# Autodesk Inventor assembly: test_rig_asmbly
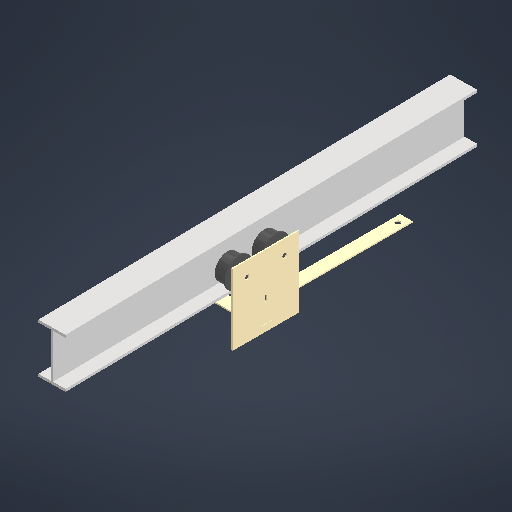
[picture p0: Inventor's stored thumbnail of the model, 512x512]
Saved by Autodesk Inventor 2027.1 (Build 311270010, 270A)
## iProperties
Created: 2026-09-04
Part Number: test_rig_asmbly
Document SubType Name: Assembly
Designer: ajrcr
Author: ajrcr
## Documents named in this file (6)
- C:\Users\ajrcr\OneDrive\Documents\Y3_s2\MCTR327\Git_Repo\Design-2026\3D parts\test_rig_asmbly.iam
- C:\Users\ajrcr\OneDrive\Documents\Y3_s2\MCTR327\Git_Repo\Design-2026\3D parts\Rail_beam.ipt
- C:\Users\ajrcr\OneDrive\Documents\Y3_s2\MCTR327\Git_Repo\Design-2026\3D parts\test_wheel_v1.ipt
- C:\Users\ajrcr\OneDrive\Documents\Y3_s2\MCTR327\Git_Repo\Design-2026\3D parts\test_rig_plate.ipt
- C:\Users\ajrcr\OneDrive\Documents\Y3_s2\MCTR327\Git_Repo\Design-2026\3D parts\rig_connector.ipt
- C:\Users\ajrcr\OneDrive\Documents\Y3_s2\MCTR327\Git_Repo\Design-2026\3D parts\rig_connector_long.ipt
## Components (10 placed, 5 different names)
1. Rail_beam:1 — Tangent:1, Tangent:2, Mate:1, Mate:2, Mate:3
2. test_wheel_v1:1 — Tangent:1, Mate:2, Mate:4
3. test_wheel_v1:2 — Mate:1, Mate:4
4. test_wheel_v1:3
5. test_wheel_v1:4
6. test_wheel_v1:5
7. test_wheel_v1:6 — Tangent:2, Mate:3
8. test_rig_plate:1 — Mate:5, Mate:6, Flush:1
9. rig_connector:1 — Mate:5, Mate:6, Flush:1
10. rig_connector_long:1
## Relationships (9: Mate 6, Tangent 2, Flush 1)
- Tangent:1: Rail_beam:1 ↔ test_wheel_v1:1
- Tangent:2: Rail_beam:1 ↔ test_wheel_v1:6
- Mate:1: Rail_beam:1 ↔ test_wheel_v1:2
- Mate:2: Rail_beam:1 ↔ test_wheel_v1:1
- Mate:3: Rail_beam:1 ↔ test_wheel_v1:6
- Mate:4 (90 mm): test_wheel_v1:1 ↔ test_wheel_v1:2
- Mate:5: test_rig_plate:1 ↔ rig_connector:1
- Mate:6: test_rig_plate:1 ↔ rig_connector:1
- Flush:1: test_rig_plate:1 ↔ rig_connector:1
## Named parameters: Finish1_Area = 575.357, Finish2_Area = 903.012, Finish3_Area = 575.357
note: some values were not read from the file. Shown as the stored number, unit unknown: "Finish1_Area", "Finish2_Area", "Finish3_Area".
